# Autodesk Inventor assembly: MP1-1001_CAM2
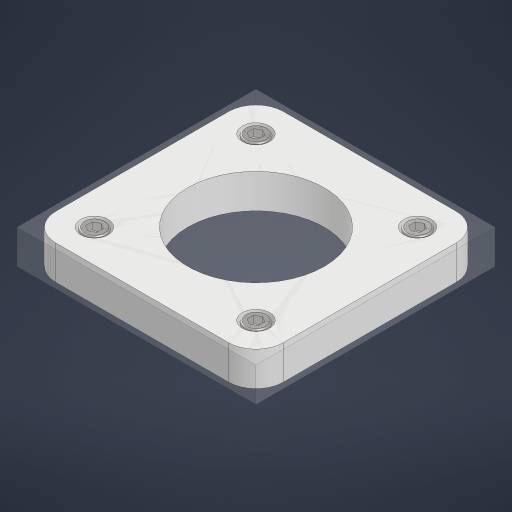
[picture p0: Inventor's stored thumbnail of the model, 512x512]
Saved by Autodesk Inventor 2024.1 (Build 281209000, 209)
## iProperties
Created: 2024-02-21
Part Number: MP1-1001_CAM2
Document SubType Name: Assembly
Designer: fablabadmin
Author: fablabadmin
## Documents named in this file (3)
- C:\Users\fablabadmin\Documents\_Benjamin_S\_3dCAD\HHVerkstad\MountPlate\_CAM\MP1-1001_CAM2.iam
- C:\Users\fablabadmin\Documents\_Benjamin_S\_3dCAD\HHVerkstad\MountPlate\MP1.iam
- C:\Users\fablabadmin\Documents\_Benjamin_S\_3dCAD\HHVerkstad\MountPlate\_CAM\SquareStock-110-110-15.ipt
## Components (2 placed, 2 different names)
1. MP1:1 [sub-assembly] — Flush:1
2. SquareStock-110-110-15:1 — Mate:1, Mate:2, Flush:1
## Relationships (3: Mate 2, Flush 1)
- Mate:1: SquareStock-110-110-15:1
- Mate:2: SquareStock-110-110-15:1
- Flush:1: MP1:1 ↔ SquareStock-110-110-15:1
